# Autodesk Inventor assembly: main
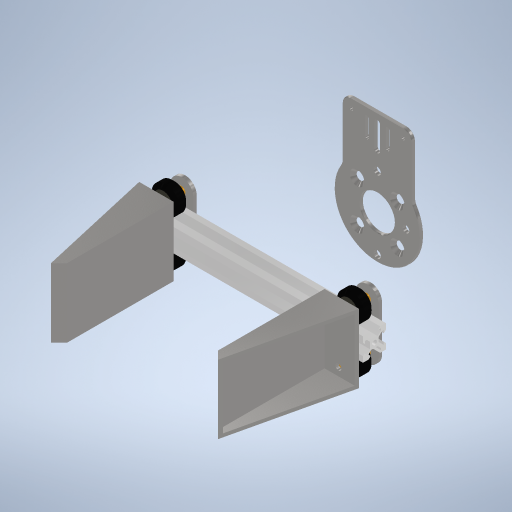
[picture p0: Inventor's stored thumbnail of the model, 512x512]
Saved by Autodesk Inventor 2024.2 (Build 282272000, 272)
## iProperties
Created: 2025-04-11
Part Number: main
Document SubType Name: Assembly
Designer: Admin
Author: Admin
## Documents named in this file (4)
- C:\Users\Admin\Documents\GitHub\GripperPropuesto\Assemblies\main.iam
- C:\Users\Admin\Documents\GitHub\GripperPropuesto\AuxiliarPieces\CameraStand\CameraStand.ipt
- C:\Users\Admin\Documents\GitHub\GripperPropuesto\Assemblies\Finger.iam
- C:\Users\Admin\Documents\GitHub\GripperPropuesto\AuxiliarPieces\AluminumProfile\AP20x20.ipt
## Components (4 placed, 3 different names)
1. CameraStand:1
2. Finger:1 [sub-assembly] — Tangent:5, Tangent:6, Tangent:7
3. Finger:2 [sub-assembly] — Tangent:1, Tangent:2, Tangent:3, Tangent:4
4. AP20x20:1 — Tangent:1, Tangent:2, Tangent:3, Tangent:4, Tangent:5, Tangent:6, Tangent:7
## Relationships (7: Tangent 7)
- Tangent:1: Finger:2 ↔ AP20x20:1
- Tangent:2: Finger:2 ↔ AP20x20:1
- Tangent:3: Finger:2 ↔ AP20x20:1
- Tangent:4: Finger:2 ↔ AP20x20:1
- Tangent:5: Finger:1 ↔ AP20x20:1
- Tangent:6: Finger:1 ↔ AP20x20:1
- Tangent:7: Finger:1 ↔ AP20x20:1
